# Autodesk Inventor assembly: Ensamble Servo + Soporte
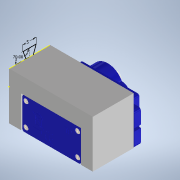
[picture p0: Inventor's stored thumbnail of the model, 180x180]
Saved by Autodesk Inventor 2020.3 (Build 243373000, 373)
## iProperties
Created: 2020-11-04
Part Number: Ensamble Servo + Soporte
Document SubType Name: Assembly
Designer: juanp
Author: juanp
## Documents named in this file (3)
- C:\Users\juanp\Desktop\Diseño EVA\Contenedores\Servo SG90\Ensamble Servo + Soporte.iam
- C:\Users\juanp\Desktop\Diseño EVA\Contenedores\Servo SG90\SG90 - Micro Servo 9g - Tower Pro.1.ipt
- C:\Users\juanp\Desktop\Diseño EVA\Contenedores\Servo SG90\Soporte Servo SG90.ipt
## Components (2 placed, 2 different names)
1. SG90 - Micro Servo 9g - Tower Pro.1:1 — Mate:1, Mate:2, Mate:3
2. Soporte Servo SG90:1 — Mate:1, Mate:2, Mate:3
## Relationships (3: Mate 3)
- Mate:1: SG90 - Micro Servo 9g - Tower Pro.1:1 ↔ Soporte Servo SG90:1
- Mate:2: SG90 - Micro Servo 9g - Tower Pro.1:1 ↔ Soporte Servo SG90:1
- Mate:3: SG90 - Micro Servo 9g - Tower Pro.1:1 ↔ Soporte Servo SG90:1
